# Autodesk Inventor assembly: Arm
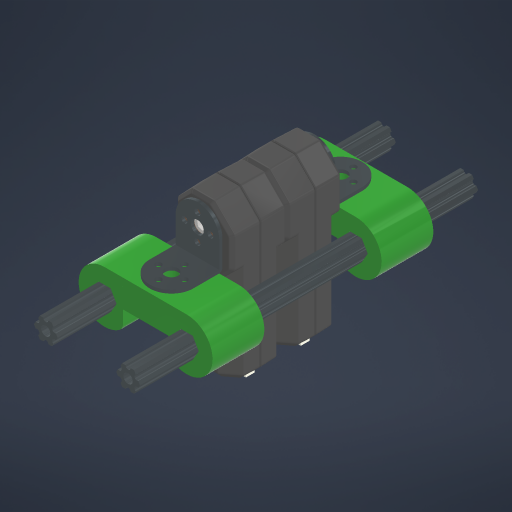
[picture p0: Inventor's stored thumbnail of the model, 512x512]
Saved by Autodesk Inventor 2024.2 (Build 282272000, 272)
## iProperties
Created: 2024-01-12
Part Number: Arm
Document SubType Name: Assembly
Designer: Allan Niles
Author: Allan Niles
## Documents named in this file (5)
- C:\Users\alniles07\Documents\Github\8400_2024_CAD\Arm.iam
- C:\Users\alniles07\Documents\Github\8400_2024_CAD\Churro Arm Mount.ipt
- C:\Users\alniles07\Documents\Github\8400_2024_CAD\Middle Churo.ipt
- C:\Users\alniles07\Documents\Github\8400_2024_CAD\Core Hex Motor.ipt
- C:\Users\alniles07\Documents\Github\8400_2024_CAD\L Bracket.ipt
## Components (8 placed, 4 different names)
1. Churro Arm Mount:1 — Mate:1, Mate:2, Mate:3, Mate:4, Mate:9, Mate:10, Flush:1
2. Churro Arm Mount:2 — Mate:5, Mate:6, Mate:11, Mate:12, Flush:2
3. Middle Churo:1 — Mate:1, Mate:2, Flush:2
4. Middle Churo:2 — Mate:3, Mate:4, Mate:5, Mate:6, Flush:1
5. Core Hex Motor:1 — Mate:7, Mate:8, Mate:14, Mate:15
6. Core Hex Motor:2 — Mate:7, Mate:8, Mate:13, Mate:16
7. L Bracket:1 — Mate:11, Mate:12, Mate:14, Mate:15
8. L Bracket:2 — Mate:9, Mate:10, Mate:13, Mate:16
## Relationships (18: Mate 16, Flush 2)
- Mate:1: Churro Arm Mount:1 ↔ Middle Churo:1
- Mate:2: Churro Arm Mount:1 ↔ Middle Churo:1
- Mate:3: Churro Arm Mount:1 ↔ Middle Churo:2
- Mate:4: Churro Arm Mount:1 ↔ Middle Churo:2
- Mate:5: Churro Arm Mount:2 ↔ Middle Churo:2
- Mate:6: Churro Arm Mount:2 ↔ Middle Churo:2
- Mate:7: Core Hex Motor:1 ↔ Core Hex Motor:2
- Mate:8: Core Hex Motor:1 ↔ Core Hex Motor:2
- Mate:9: Churro Arm Mount:1 ↔ L Bracket:2
- Mate:10: Churro Arm Mount:1 ↔ L Bracket:2
- Mate:11: Churro Arm Mount:2 ↔ L Bracket:1
- Mate:12: Churro Arm Mount:2 ↔ L Bracket:1
- Mate:13: Core Hex Motor:2 ↔ L Bracket:2
- Mate:14: Core Hex Motor:1 ↔ L Bracket:1
- Mate:15: Core Hex Motor:1 ↔ L Bracket:1
- Mate:16: Core Hex Motor:2 ↔ L Bracket:2
- Flush:1 (-36.3093 mm): Churro Arm Mount:1 ↔ Middle Churo:2
- Flush:2 (36.3093 mm): Churro Arm Mount:2 ↔ Middle Churo:1
